# Autodesk Inventor assembly: NonrebreathAsm
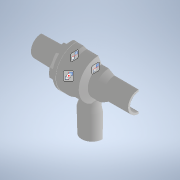
[picture p0: Inventor's stored thumbnail of the model, 180x180]
Saved by Autodesk Inventor 2020 (Build 240168000, 168)
## iProperties
Created: 2020-06-04
Part Number: NonrebreathAsm
Document SubType Name: Assembly
Designer: Theo Cominotto
Author: Theo Cominotto
## Documents named in this file (5)
- C:\Users\Theo Cominotto\Dropbox\Beademingstoestel VUB\Beademingstoestel VUB-PEEP VALVE\Archive - Old Cad files\NonrebreathAsm.iam
- C:\Users\Theo Cominotto\Dropbox\Beademingstoestel VUB\Beademingstoestel VUB-PEEP VALVE\Archive - Old Cad files\Nonrebreath_Bottom.ipt
- C:\Users\Theo Cominotto\Dropbox\Beademingstoestel VUB\Beademingstoestel VUB-PEEP VALVE\3D print set -FDM-V2\02-ExpTopTaper.ipt
- C:\Users\Theo Cominotto\Dropbox\Beademingstoestel VUB\Beademingstoestel VUB-PEEP VALVE\Archive - Old Cad files\ExpSeal.ipt
- C:\Users\Theo Cominotto\Dropbox\Beademingstoestel VUB\Beademingstoestel VUB-PEEP VALVE\Archive - Old Cad files\Umbrella valve\rubber replica_Model_DONOTUSE.ipt
## Components (4 placed, 4 different names)
1. Nonrebreath_Bottom:1 — Mate:1, Mate:3, Mate:5, Mate:6, Mate:7
2. 02-ExpTopTaper:1 — Mate:1, Mate:2, Mate:4, Mate:8
3. ExpSeal:1 — Mate:2, Mate:3, Mate:4
4. rubber replica_Model_DONOTUSE:1 — Mate:7, Mate:8
## Relationships (8: Mate 8)
- Mate:1: Nonrebreath_Bottom:1 ↔ 02-ExpTopTaper:1
- Mate:2: 02-ExpTopTaper:1 ↔ ExpSeal:1
- Mate:3: Nonrebreath_Bottom:1 ↔ ExpSeal:1
- Mate:4 (-0.5 mm): 02-ExpTopTaper:1 ↔ ExpSeal:1
- Mate:5: Nonrebreath_Bottom:1
- Mate:6: Nonrebreath_Bottom:1
- Mate:7: Nonrebreath_Bottom:1 ↔ rubber replica_Model_DONOTUSE:1
- Mate:8: 02-ExpTopTaper:1 ↔ rubber replica_Model_DONOTUSE:1
